# Autodesk Inventor assembly: Assembly2
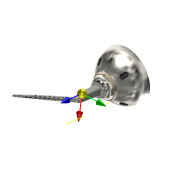
[picture p0: Inventor's stored thumbnail of the model, 180x180]
Saved by Autodesk Inventor 2018 (Build 220112000, 112)
## iProperties
Created: 2018-11-29
Part Number: Assembly2
Document SubType Name: Assembly
Designer: Ousama
Author: Ousama
## Documents named in this file (5)
- C:\Users\Ousama\Desktop\McMaster\IBEHS 1P10A\DP-2\CAD model\Final parts\Assembly2.iam
- C:\Users\Ousama\Desktop\McMaster\IBEHS 1P10A\DP-2\CAD model\Final parts\Femoral Head DP-2.ipt
- C:\Users\Ousama\Desktop\McMaster\IBEHS 1P10A\DP-2\CAD model\Final parts\Liner 2.ipt
- C:\Users\Ousama\Desktop\McMaster\IBEHS 1P10A\DP-2\CAD model\Final parts\Stem 2.ipt
- C:\Users\Ousama\Desktop\McMaster\IBEHS 1P10A\DP-2\CAD model\Final parts\AcetabulumCup DP-2.ipt
## Components (4 placed, 4 different names)
1. Femoral Head DP-2:1 — Ball:1, Mate:1, Rigid:2
2. Liner 2:1 — Ball:1, Rigid:1
3. Stem 2:1 — Mate:1, Rigid:2
4. AcetabulumCup DP-2:1 — Rigid:1
## Relationships (4: WeldJoint 2, BallJoint 1, Mate 1)
- Ball:1: Femoral Head DP-2:1 ↔ Liner 2:1
- Mate:1: Femoral Head DP-2:1 ↔ Stem 2:1
- Rigid:1 [WeldJoint]: Liner 2:1 ↔ AcetabulumCup DP-2:1
- Rigid:2 [WeldJoint]: Femoral Head DP-2:1 ↔ Stem 2:1
